# Autodesk Inventor assembly: Ensamble Lab Dinamica - Luis Lopez - 1175719
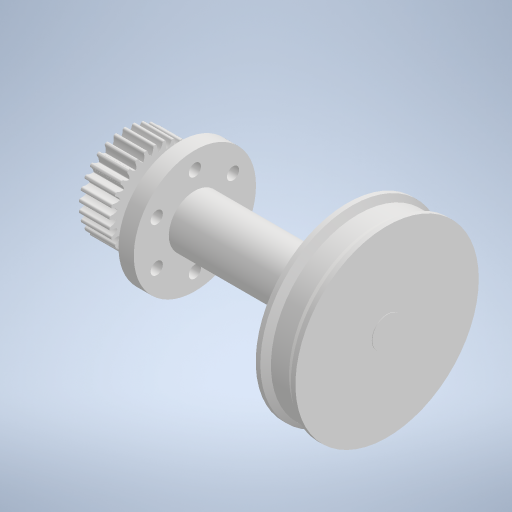
[picture p0: Inventor's stored thumbnail of the model, 512x512]
Saved by Autodesk Inventor 2024.2 (Build 282272000, 272)
## iProperties
Created: 2024-03-30
Part Number: Ensamble Lab Dinamica - Luis Lopez - 1175719
Document SubType Name: Assembly
Designer: luisf
Author: luisf
## Documents named in this file (3)
- C:\Users\luisf\Downloads\Ensamble Lab Dinamica - Luis Lopez - 1175719.iam
- C:\Users\luisf\Downloads\Ensamble Laboratorio - Luis Lopez.iam
- C:\Users\luisf\Downloads\RODADURA NUEVA 222.ipt
## Components (2 placed, 2 different names)
1. Ensamble Laboratorio - Luis Lopez:1 [sub-assembly] — Rotational:1
2. RODADURA NUEVA 222:1 — Rotational:1
## Relationships (1: RevoluteJoint 1)
- Rotational:1 [RevoluteJoint]: Ensamble Laboratorio - Luis Lopez:1 ↔ RODADURA NUEVA 222:1
